# Autodesk Inventor assembly: S16x1
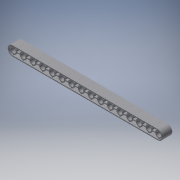
[picture p0: Inventor's stored thumbnail of the model, 180x180]
Saved by Autodesk Inventor 2019 (Build 230136000, 136)
## iProperties
Created: 2019-01-31
Part Number: S16x1
Document SubType Name: Assembly
Designer: Varga Daniel
Author: Varga Daniel
## Documents named in this file (4)
- C:\!_Dani\!_cloud\OneDrive\!_munka\Revolution\RevvyDemoKit\Structural parts\Straight Beams\S3+x1\S16x1.iam
- C:\!_Dani\!_cloud\OneDrive\!_munka\Revolution\RevvyDemoKit\Structural parts\Straight Beams\straight_beam_single_end_part.ipt
- C:\!_Dani\!_cloud\OneDrive\!_munka\Revolution\RevvyDemoKit\Structural parts\Straight Beams\straight_beam_single_inner_part.ipt
- C:\!_Dani\!_cloud\OneDrive\!_munka\Revolution\RevvyDemoKit\Structural parts\Straight Beams\S3+x1.iam
## Components (16 placed, 2 different names)
1. straight_beam_single_end_part:1 — Flush:1, Flush:2, Mate:1, Flush:3, Flush:4, Mate:2
2. straight_beam_single_end_part:2 — Flush:1, Flush:2, Mate:1
3. straight_beam_single_inner_part:1 — Flush:3, Flush:4, Mate:2
4. straight_beam_single_inner_part:2
5. straight_beam_single_inner_part:3
6. straight_beam_single_inner_part:4
7. straight_beam_single_inner_part:5
8. straight_beam_single_inner_part:6
9. straight_beam_single_inner_part:7
10. straight_beam_single_inner_part:8
11. straight_beam_single_inner_part:9
12. straight_beam_single_inner_part:10
13. straight_beam_single_inner_part:11
14. straight_beam_single_inner_part:12
15. straight_beam_single_inner_part:13
16. straight_beam_single_inner_part:14
## Component patterns: (14 elements, first: straight_beam_single_inner_part:1)
## Relationships (6: Flush 4, Mate 2)
- Flush:1: straight_beam_single_end_part:1 ↔ straight_beam_single_end_part:2
- Flush:2: straight_beam_single_end_part:1 ↔ straight_beam_single_end_part:2
- Mate:1 (140 mm): straight_beam_single_end_part:1 ↔ straight_beam_single_end_part:2
- Flush:3: straight_beam_single_end_part:1 ↔ straight_beam_single_inner_part:1
- Flush:4: straight_beam_single_end_part:1 ↔ straight_beam_single_inner_part:1
- Mate:2: straight_beam_single_end_part:1 ↔ straight_beam_single_inner_part:1
